# Autodesk Inventor assembly: Roller Shaft
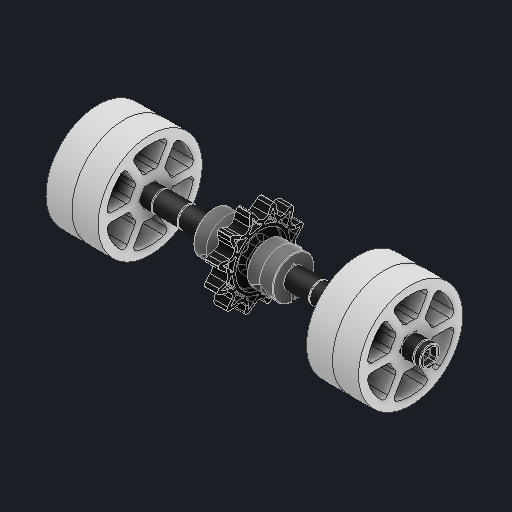
[picture p0: Inventor's stored thumbnail of the model, 512x512]
Saved by Autodesk Inventor 2025 (Build 290162000, 162)
## iProperties
Created: 2024-10-20
Part Number: Roller Shaft
Document SubType Name: Assembly
Designer: Averey Ku
Author: Averey Ku
## Documents named in this file (11)
- D:\VEX\High Stakes\CAD\V2\Hook\Roller Shaft.iam
- D:\VEX\High Stakes\CAD\ROBOPROS-CAD-Inventor\Motion\Sprockets\9P Sprocket\9P 12T Sprocket, No Insert.iam
- D:\VEX\High Stakes\CAD\ROBOPROS-CAD-Inventor\Motion\Sprockets\9P Sprocket.iam
- D:\VEX\High Stakes\CAD\ROBOPROS-CAD-Inventor\Motion\Wheels\Flex Wheels\2.000 Flex Wheel\2.000 30A .500.ipt
- D:\VEX\High Stakes\CAD\ROBOPROS-CAD-Inventor\Motion\Wheels\Flex Wheels\2.000 Flex Wheel.ipt
- D:\VEX\High Stakes\CAD\ROBOPROS-CAD-Inventor\Motion\Shaft HS\HS Shaft Collar.ipt
- D:\VEX\High Stakes\CAD\ROBOPROS-CAD-Inventor\Motion\Shaft HS\HS Spacer\HSpacer .2500.ipt
- D:\VEX\High Stakes\CAD\ROBOPROS-CAD-Inventor\Motion\Shaft HS\HS Spacer.ipt
- D:\VEX\High Stakes\CAD\ROBOPROS-CAD-Inventor\Motion\Shaft HS\HS Spacer\HSpacer .5000.ipt
- D:\VEX\High Stakes\CAD\ROBOPROS-CAD-Inventor\Motion\Shaft HS\HS Spacer\HSpacer .0625.ipt
- D:\VEX\High Stakes\CAD\ROBOPROS-CAD-Inventor\Motion\Shaft HS\HS Spacer\HSpacer .1250.ipt
## Components (17 placed, 7 different names)
1. 9P 12T Sprocket, No Insert:1 [sub-assembly]
2. 2.000 30A .500:1
3. 2.000 30A .500:2 — Insert:15
4. 2.000 30A .500:3 — Insert:16
5. 2.000 30A .500:4
6. HS Shaft Collar:1 — Mate:2
7. HSpacer .2500:1
8. HSpacer .5000:2 — Mate:3, Mate:4
9. HSpacer .5000:3
10. HS Shaft Collar:2
11. HSpacer .2500:4
12. HSpacer .5000:5
13. HSpacer .5000:6
14. HSpacer .0625:7 — Insert:13
15. HSpacer .2500:8 — Insert:13, Insert:16
16. HSpacer .2500:10 — Insert:15, Insert:17
17. HSpacer .1250:11 — Insert:17
## Relationships (20: Insert 16, Mate 4)
- [Insert]: 2.000 30A .500:1 ↔ 2.000 30A .500:2
- [Insert]: 2.000 30A .500:3 ↔ 2.000 30A .500:4
- [Insert] (-152.4 mm): 2.000 30A .500:2 ↔ 2.000 30A .500:3
- [Mate]: 9P 12T Sprocket, No Insert:1 ↔ 2.000 30A .500:1
- [Insert] (44.45 mm): 9P 12T Sprocket, No Insert:1 ↔ 2.000 30A .500:1
- [Insert]: 9P 12T Sprocket, No Insert:1 ↔ HS Shaft Collar:1
- [Insert]: HS Shaft Collar:1 ↔ HSpacer .5000:2
- [Insert]: HSpacer .5000:2 ↔ HSpacer .5000:3
- [Insert]: HSpacer .2500:1 ↔ HSpacer .5000:3
- [Insert]: HS Shaft Collar:2 ↔ HSpacer .5000:5
- [Insert]: HSpacer .5000:5 ↔ HSpacer .5000:6
- [Insert]: HSpacer .2500:4 ↔ HSpacer .5000:6
- [Insert]: 9P 12T Sprocket, No Insert:1 ↔ HS Shaft Collar:2
- Mate:2 (6.35 mm): HS Shaft Collar:1
- Mate:3: HSpacer .5000:2
- Mate:4: HSpacer .5000:2
- Insert:13: HSpacer .0625:7 ↔ HSpacer .2500:8
- Insert:15: 2.000 30A .500:2 ↔ HSpacer .2500:10
- Insert:16: 2.000 30A .500:3 ↔ HSpacer .2500:8
- Insert:17: HSpacer .2500:10 ↔ HSpacer .1250:11
## Named parameters: d61_d58 = 0 mm, d62_d59 = 0 mm, d63_d60 = 0 mm, d42_d40 = 0 mm
